# Autodesk Inventor assembly: banhxe
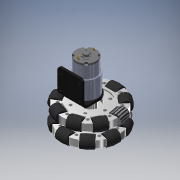
[picture p0: Inventor's stored thumbnail of the model, 180x180]
Saved by Autodesk Inventor 2019 (Build 230136000, 136)
## iProperties
Created: 2021-01-09
Part Number: banhxe
Document SubType Name: Assembly
Designer: Admin
Author: Admin
## Documents named in this file (4)
- C:\Users\Admin\Documents\Inventor\Doan\banhxe.iam
- C:\Users\Admin\Documents\Inventor\Doan\DualOmniWithHub1.iam
- C:\Users\Admin\Documents\Inventor\Doan\JGB37-520.iam
- C:\Users\Admin\Documents\Inventor\Doan\JGB37-520 12 v metal geared motor bracket.ipt
## Components (3 placed, 3 different names)
1. DualOmniWithHub1:1 [sub-assembly] — Mate:4, Mate:5
2. JGB37-520:1 [sub-assembly] — Mate:1, Mate:2, Mate:3, Mate:4, Mate:5
3. JGB37-520 12 v metal geared motor bracket:1 — Mate:1, Mate:2, Mate:3
## Relationships (5: Mate 5)
- Mate:1: JGB37-520:1 ↔ JGB37-520 12 v metal geared motor bracket:1
- Mate:2: JGB37-520:1 ↔ JGB37-520 12 v metal geared motor bracket:1
- Mate:3: JGB37-520:1 ↔ JGB37-520 12 v metal geared motor bracket:1
- Mate:4: DualOmniWithHub1:1 ↔ JGB37-520:1
- Mate:5: DualOmniWithHub1:1 ↔ JGB37-520:1
